# Autodesk Inventor assembly: Celda_reposabrasos
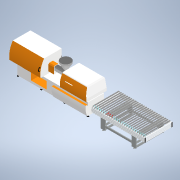
[picture p0: Inventor's stored thumbnail of the model, 180x180]
Saved by Autodesk Inventor 2022 (Build 260153000, 153)
## iProperties
Created: 2022-06-19
Part Number: Celda_reposabrasos
Document SubType Name: Assembly
Designer: Yeison
Author: Yeison
## Documents named in this file (3)
- C:\Users\Yeison\Documents\GitHub\SediaAutomatica\6 - Digital Factory\Modelos\Estacion de inyeccion de reposabrazos\Celda_reposabrasos.iam
- C:\Users\Yeison\Documents\GitHub\SediaAutomatica\6 - Digital Factory\Modelos\Conveyor\Line shaft roller conveyor_100.ipt
- C:\Users\Yeison\Documents\GitHub\SediaAutomatica\6 - Digital Factory\Modelos\Máquina de moldeo por inyección\Injection_molding_100.ipt
## Components (2 placed, 2 different names)
1. Line shaft roller conveyor_100:1 — Flush:1, Flush:2
2. Injection_molding_100:1 — Flush:1, Flush:2
## Relationships (2: Flush 2)
- Flush:1: Line shaft roller conveyor_100:1 ↔ Injection_molding_100:1
- Flush:2 (2.54 mm): Line shaft roller conveyor_100:1 ↔ Injection_molding_100:1
